# Autodesk Inventor assembly: Odom_assembly_test
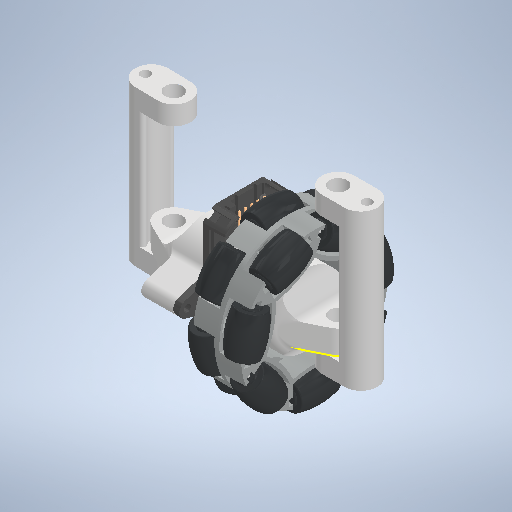
[picture p0: Inventor's stored thumbnail of the model, 512x512]
Saved by Autodesk Inventor 2025.1 (Build 291241020, 241B)
## iProperties
Created: 2024-11-14
Part Number: Odom_assembly_test
Document SubType Name: Assembly
Designer: AtuStem
Author: AtuStem
## Documents named in this file (6)
- C:\Users\AtuStem\Documents\GitHub\ATUM-V5RC-High-Stakes-CAD\Protobot\Odom_assembly_test.iam
- C:\Users\AtuStem\Documents\GitHub\ATUM-V5RC-High-Stakes-CAD\Odometer_Test_Bracket.ipt
- C:\Users\AtuStem\Documents\GitHub\ATUM-V5RC-High-Stakes-CAD\Protobot\Odom_Part1_Encoder.ipt
- C:\Users\AtuStem\Documents\GitHub\ATUM-V5RC-High-Stakes-CAD\Same_Sky_AMT102-0048-N2000-W (1)\Same_Sky_AMT102-0048-N2000-W.iam
- C:\Users\AtuStem\Documents\GitHub\ATUM-V5RC-High-Stakes-CAD\Protobot\Odom_Part1.ipt
- C:\Users\AtuStem\Documents\GitHub\ATUM-V5RC-High-Stakes-CAD\Protobot\IQ_OMNI.iam
## Components (6 placed, 5 different names)
1. Odom_Part1_Encoder:1 — Mate:3, Mate:4, Mate:5, Mate:10, Mate:13, Mate:15
2. Same_Sky_AMT102-0048-N2000-W:1 [sub-assembly] — Mate:3, Mate:4, Mate:5
3. Odom_Part1:1 — Mate:10, Mate:11, Mate:12, Mate:14
4. IQ_OMNI:1 [sub-assembly] — Mate:11, Mate:12
5. Odometer_Test_Bracket:1 — Mate:13, Flush:1, Mate:15
6. Odometer_Test_Bracket:2 — Mate:14, Flush:1
## Relationships (10: Mate 9, Flush 1)
- Mate:3: Odom_Part1_Encoder:1 ↔ Same_Sky_AMT102-0048-N2000-W:1
- Mate:4: Odom_Part1_Encoder:1 ↔ Same_Sky_AMT102-0048-N2000-W:1
- Mate:5: Odom_Part1_Encoder:1 ↔ Same_Sky_AMT102-0048-N2000-W:1
- Mate:10: Odom_Part1_Encoder:1 ↔ Odom_Part1:1
- Mate:11: Odom_Part1:1 ↔ IQ_OMNI:1
- Mate:12: Odom_Part1:1 ↔ IQ_OMNI:1
- Mate:13: Odom_Part1_Encoder:1 ↔ Odometer_Test_Bracket:1
- Mate:14: Odom_Part1:1 ↔ Odometer_Test_Bracket:2
- Flush:1: Odometer_Test_Bracket:1 ↔ Odometer_Test_Bracket:2
- Mate:15: Odom_Part1_Encoder:1 ↔ Odometer_Test_Bracket:1
